# Autodesk Inventor assembly: Montagem1
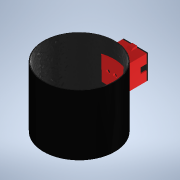
[picture p0: Inventor's stored thumbnail of the model, 180x180]
Saved by Autodesk Inventor 2022 (Build 260153000, 153)
## iProperties
Created: 2024-02-25
Part Number: Montagem1
Document SubType Name: Assembly
Designer: Daniel
Author: Daniel
## Documents named in this file (4)
- C:\Users\Daniel\Documents\Inventor\prototipo2_V3\Montagem1.iam
- C:\Users\Daniel\Documents\Inventor\prototipo2_V3\caixaled_pt1.ipt
- C:\Users\Daniel\Documents\Inventor\prototipo2_V3\caixaled_pt2.ipt
- C:\Users\Daniel\Documents\Inventor\prototipo2_V3\velcro.ipt
## Components (3 placed, 3 different names)
1. caixaled_pt1:1 — Alinhado:1, Alinhado:2, Coincidente:2
2. caixaled_pt2:1 — Alinhado:1, Alinhado:2, Coincidente:2
3. velcro:1
## Relationships (3: Flush 2, Mate 1)
- Alinhado:1 [Flush]: caixaled_pt1:1 ↔ caixaled_pt2:1
- Alinhado:2 [Flush]: caixaled_pt1:1 ↔ caixaled_pt2:1
- Coincidente:2 [Mate]: caixaled_pt1:1 ↔ caixaled_pt2:1
